# Autodesk Inventor assembly: Assembly1
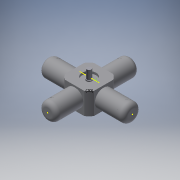
[picture p0: Inventor's stored thumbnail of the model, 180x180]
Saved by Autodesk Inventor 2018 (Build 220112000, 112)
## iProperties
Created: 2018-11-06
Part Number: Assembly1
Document SubType Name: Assembly
Designer: HP
Author: HP
## Documents named in this file (10)
- C:\Users\HP\Documents\MCP100\motor\Assembly1.iam
- C:\Users\HP\Documents\MCP100\motor\cylinder.ipt
- C:\Users\HP\Documents\MCP100\motor\cylinder_head.ipt
- C:\Users\HP\Documents\MCP100\motor\hub.ipt
- C:\Users\HP\Documents\MCP100\motor\crank.ipt
- C:\Users\HP\Documents\MCP100\motor\cam_shaft.ipt
- C:\Users\HP\Documents\MCP100\motor\connecting_link.ipt
- C:\Users\HP\Documents\MCP100\motor\bearing.ipt
- C:\Users\HP\Documents\MCP100\motor\gauge_pin.ipt
- C:\Users\HP\Documents\MCP100\motor\piston.ipt
## Components (25 placed, 9 different names)
1. cylinder:1 — Rigid:3, Rigid:5, Angle:1, Cylindrical:1
2. cylinder_head:1 — Rigid:3
3. cylinder:2 — Rigid:2, Rigid:6
4. cylinder_head:2 — Rigid:2, Angle:3, Mate:4
5. cylinder:3 — Rigid:1, Rigid:8
6. cylinder_head:3 — Rigid:1, Angle:4, Mate:6
7. cylinder:4 — Rigid:4, Rigid:7
8. cylinder_head:4 — Rigid:4, Angle:2, Mate:2
9. hub:1 — Rigid:5, Rigid:6, Rigid:7, Rigid:8, Rotational:16
10. crank:1 — Rotational:1, Flush:1, Rotational:16
11. cam_shaft:1 — Rotational:1, Rotational:2, Rotational:3, Rotational:4, Rotational:5, Rotational:6, Rotational:7, Rotational:8, Mate:5
12. connecting_link:1 — Rotational:4, Rotational:10, Mate:1
13. connecting_link:2 — Rotational:3, Rotational:11
14. connecting_link:3 — Rotational:2, Rotational:9
15. bearing:1 — Rotational:6
16. bearing:2 — Rotational:7
17. bearing:3 — Rotational:5
18. gauge_pin:1 — Rotational:11, Mate:3
19. gauge_pin:2 — Rotational:9, Mate:7
20. gauge_pin:3 — Rotational:8
21. gauge_pin:4 — Rotational:10
22. piston:1 — Angle:2, Mate:2, Mate:3
23. piston:2 — Angle:4, Mate:6, Mate:7
24. piston:3 — Angle:1, Cylindrical:1, Mate:1
25. piston:4 — Angle:3, Mate:4, Mate:5
## Relationships (33: RevoluteJoint 12, WeldJoint 8, Mate 7, Angle 4, Flush 1, CylindricalJoint 1)
- Rigid:1 [WeldJoint]: cylinder:3 ↔ cylinder_head:3
- Rigid:2 [WeldJoint]: cylinder:2 ↔ cylinder_head:2
- Rigid:3 [WeldJoint]: cylinder:1 ↔ cylinder_head:1
- Rigid:4 [WeldJoint]: cylinder:4 ↔ cylinder_head:4
- Rigid:5 [WeldJoint]: cylinder:1 ↔ hub:1
- Rigid:6 [WeldJoint]: cylinder:2 ↔ hub:1
- Rigid:7 [WeldJoint]: cylinder:4 ↔ hub:1
- Rigid:8 [WeldJoint]: cylinder:3 ↔ hub:1
- Rotational:1 [RevoluteJoint]: crank:1 ↔ cam_shaft:1
- Rotational:2 [RevoluteJoint]: cam_shaft:1 ↔ connecting_link:3
- Rotational:3 [RevoluteJoint]: cam_shaft:1 ↔ connecting_link:2
- Rotational:4 [RevoluteJoint]: cam_shaft:1 ↔ connecting_link:1
- Rotational:5 [RevoluteJoint]: cam_shaft:1 ↔ bearing:3
- Rotational:6 [RevoluteJoint]: cam_shaft:1 ↔ bearing:1
- Rotational:7 [RevoluteJoint]: cam_shaft:1 ↔ bearing:2
- Rotational:8 [RevoluteJoint]: cam_shaft:1 ↔ gauge_pin:3
- Rotational:9 [RevoluteJoint]: connecting_link:3 ↔ gauge_pin:2
- Rotational:10 [RevoluteJoint]: connecting_link:1 ↔ gauge_pin:4
- Rotational:11 [RevoluteJoint]: connecting_link:2 ↔ gauge_pin:1
- Flush:1: crank:1
- Rotational:16 [RevoluteJoint]: hub:1 ↔ crank:1
- Angle:1 (0 deg): cylinder:1 ↔ piston:3
- Cylindrical:1: cylinder:1 ↔ piston:3
- Mate:1: connecting_link:1 ↔ piston:3
- Angle:2 (180 deg): cylinder_head:4 ↔ piston:1
- Mate:2: cylinder_head:4 ↔ piston:1
- Mate:3: gauge_pin:1 ↔ piston:1
- Angle:3 (180 deg): cylinder_head:2 ↔ piston:4
- Mate:4: cylinder_head:2 ↔ piston:4
- Mate:5: cam_shaft:1 ↔ piston:4
- Angle:4 (180 deg): cylinder_head:3 ↔ piston:2
- Mate:6: cylinder_head:3 ↔ piston:2
- Mate:7: gauge_pin:2 ↔ piston:2
